# Autodesk Inventor assembly: NEMA 17
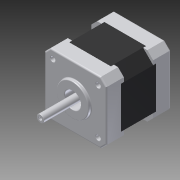
[picture p0: Inventor's stored thumbnail of the model, 180x180]
Saved by Autodesk Inventor 2015 (Build 190159000, 159)
## iProperties
Created: 2017-01-16
Part Number: NEMA 17
Document SubType Name: Assembly
Designer: Ernest
Sending System: SolidWorks 2012
Last Author: ELECTRO
Author: Ernest
## Documents named in this file (5)
- C:\Users\Ernest\Documents\Capstone-Project\doc\CAD\Imported Components\NEMA 17.iam
- C:\Users\Ernest\Downloads\Imported Components\Imported Components\NEMA 17\Base.ipt
- C:\Users\Ernest\Downloads\Imported Components\Imported Components\NEMA 17\Cuerpo.ipt
- C:\Users\Ernest\Downloads\Imported Components\Imported Components\NEMA 17\Tapa.ipt
- C:\Users\Ernest\Downloads\Imported Components\Imported Components\NEMA 17\Eje.ipt
## Components (4 placed, 4 different names)
1. Base:1 — Mate:1, Flush:1, Mate:2, Flush:2, Flush:3, Flush:4, Mate:4
2. Cuerpo:1 — Flush:3, Flush:4, Mate:4
3. Tapa:1 — Mate:1, Mate:3, Flush:2
4. Eje:1 — Flush:1, Mate:2, Mate:3
## Relationships (8: Mate 4, Flush 4)
- Mate:1 (-44 mm): Base:1 ↔ Tapa:1
- Flush:1: Base:1 ↔ Eje:1
- Mate:2: Base:1 ↔ Eje:1
- Mate:3: Tapa:1 ↔ Eje:1
- Flush:2: Base:1 ↔ Tapa:1
- Flush:3: Base:1 ↔ Cuerpo:1
- Flush:4: Base:1 ↔ Cuerpo:1
- Mate:4: Base:1 ↔ Cuerpo:1
